# Autodesk Inventor assembly: pcb_assembly
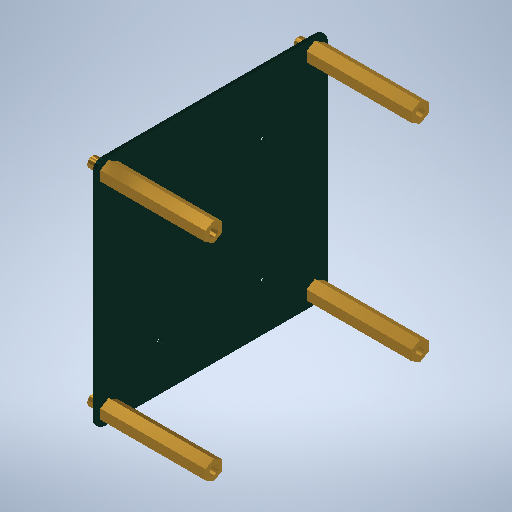
[picture p0: Inventor's stored thumbnail of the model, 512x512]
Saved by Autodesk Inventor 2025.1 (Build 291241000, 241)
## iProperties
Created: 2022-11-08
Part Number: pcb_assembly
Document SubType Name: Assembly
Designer: Thomas
Author: Thomas
## Documents named in this file (3)
- C:\Users\baince\Documents\Cours\Ateliers ROB\Autodesk Inventor\Car_Assemblage\Export_Prof\pcb_assembly.iam
- C:\Users\baince\Documents\Cours\Ateliers ROB\Autodesk Inventor\Car_Assemblage\Export_Prof\pcb.ipt
- C:\Users\baince\Documents\Cours\Ateliers ROB\Autodesk Inventor\Car_2023_Prof_12-10-2023\Workspaces\Espace de travail\Entretoise-M5-50_806-6651.ipt
## Components (5 placed, 2 different names)
1. pcb:1 — Mate:4, Mate:5, Mate:6, Mate:7, Mate:8, Mate:9, Mate:10, Mate:11
2. Entretoise-M5-50_806-6651:1 — Mate:4, Mate:5
3. Entretoise-M5-50_806-6651:2 — Mate:6, Mate:11
4. Entretoise-M5-50_806-6651:3 — Mate:7, Mate:10
5. Entretoise-M5-50_806-6651:4 — Mate:8, Mate:9
## Relationships (8: Mate 8)
- Mate:4: pcb:1 ↔ Entretoise-M5-50_806-6651:1
- Mate:5: pcb:1 ↔ Entretoise-M5-50_806-6651:1
- Mate:6: pcb:1 ↔ Entretoise-M5-50_806-6651:2
- Mate:7: pcb:1 ↔ Entretoise-M5-50_806-6651:3
- Mate:8: pcb:1 ↔ Entretoise-M5-50_806-6651:4
- Mate:9: pcb:1 ↔ Entretoise-M5-50_806-6651:4
- Mate:10: pcb:1 ↔ Entretoise-M5-50_806-6651:3
- Mate:11: pcb:1 ↔ Entretoise-M5-50_806-6651:2
